# Autodesk Inventor assembly: Team_2374
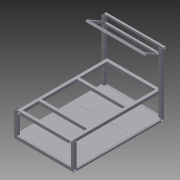
[picture p0: Inventor's stored thumbnail of the model, 180x180]
Saved by Autodesk Inventor 2012 (Build 160160000, 160)
## iProperties
Created: 2011-10-19
Part Number: Team_2374
Document SubType Name: Assembly
Designer: Ian Walters
Mass: 25411.4 g
Surface Area: 59424.9 cm^2
Volume: 9376.89 cm^3
Density: 2.71 g/cm^3
_SolveAssemblyDoc: Frame Generator Solve Assembly
_Version: 15.0.0
Author: Ian Walters
## Documents named in this file (5)
- C:\Users\Ian Walters\Dropbox\CAD Inventor\Preseason Projects\Cart Competition Cart\Team 2374\Team_2374.iam
- C:\Users\Ian Walters\Dropbox\CAD Inventor\Preseason Projects\Cart Competition Cart\Team 2374\Cart Skeleton.ipt
- C:\Users\Ian Walters\Dropbox\CAD Inventor\Preseason Projects\Cart Competition Cart\Team 2374\Team_2374\Frame\Cart Frame.iam
- C:\Users\Ian Walters\Dropbox\CAD Inventor\Preseason Projects\Cart Competition Cart\Team 2374\Bottom Sheet.ipt
- C:\Users\Ian Walters\Dropbox\CAD Inventor\Preseason Projects\Cart Competition Cart\Team 2374\IFI 114 - .1875 x 0.25.ipt
## Components (111 placed, 4 different names)
1. Cart Skeleton:1
2. Cart Frame:1 [sub-assembly] — Mate:1, Mate:2, Mate:3
3. Bottom Sheet:1 — Mate:1, Mate:2, Mate:3, Insert:1, Insert:2, Insert:3, Insert:4
4. IFI 114 - .1875 x 0.25:1 — Insert:1
5. IFI 114 - .1875 x 0.25:2 — Insert:2
6. IFI 114 - .1875 x 0.25:3 — Insert:3
7. IFI 114 - .1875 x 0.25:4 — Insert:4
8. IFI 114 - .1875 x 0.25:5
9. IFI 114 - .1875 x 0.25:6
10. IFI 114 - .1875 x 0.25:7
11. IFI 114 - .1875 x 0.25:8
12. IFI 114 - .1875 x 0.25:9
13. IFI 114 - .1875 x 0.25:10
14. IFI 114 - .1875 x 0.25:11
15. IFI 114 - .1875 x 0.25:12
16. IFI 114 - .1875 x 0.25:13
17. IFI 114 - .1875 x 0.25:14
18. IFI 114 - .1875 x 0.25:15
19. IFI 114 - .1875 x 0.25:16
20. IFI 114 - .1875 x 0.25:17
21. IFI 114 - .1875 x 0.25:18
22. IFI 114 - .1875 x 0.25:19
23. IFI 114 - .1875 x 0.25:20
24. IFI 114 - .1875 x 0.25:21
25. IFI 114 - .1875 x 0.25:22
26. IFI 114 - .1875 x 0.25:23
27. IFI 114 - .1875 x 0.25:24
28. IFI 114 - .1875 x 0.25:25
29. IFI 114 - .1875 x 0.25:26
30. IFI 114 - .1875 x 0.25:27
31. IFI 114 - .1875 x 0.25:28
32. IFI 114 - .1875 x 0.25:29
33. IFI 114 - .1875 x 0.25:30
34. IFI 114 - .1875 x 0.25:31
35. IFI 114 - .1875 x 0.25:32
36. IFI 114 - .1875 x 0.25:33
37. IFI 114 - .1875 x 0.25:34
38. IFI 114 - .1875 x 0.25:35
39. IFI 114 - .1875 x 0.25:36
40. IFI 114 - .1875 x 0.25:37
41. IFI 114 - .1875 x 0.25:38
42. IFI 114 - .1875 x 0.25:39
43. IFI 114 - .1875 x 0.25:40
44. IFI 114 - .1875 x 0.25:41
45. IFI 114 - .1875 x 0.25:42
46. IFI 114 - .1875 x 0.25:43
47. IFI 114 - .1875 x 0.25:44
48. IFI 114 - .1875 x 0.25:45
49. IFI 114 - .1875 x 0.25:46
50. IFI 114 - .1875 x 0.25:47
51. IFI 114 - .1875 x 0.25:48
52. IFI 114 - .1875 x 0.25:49
53. IFI 114 - .1875 x 0.25:50
54. IFI 114 - .1875 x 0.25:51
55. IFI 114 - .1875 x 0.25:52
56. IFI 114 - .1875 x 0.25:53
57. IFI 114 - .1875 x 0.25:54
58. IFI 114 - .1875 x 0.25:55
59. IFI 114 - .1875 x 0.25:56
60. IFI 114 - .1875 x 0.25:57
61. IFI 114 - .1875 x 0.25:58
62. IFI 114 - .1875 x 0.25:59
63. IFI 114 - .1875 x 0.25:60
64. IFI 114 - .1875 x 0.25:61
65. IFI 114 - .1875 x 0.25:62
66. IFI 114 - .1875 x 0.25:63
67. IFI 114 - .1875 x 0.25:64
68. IFI 114 - .1875 x 0.25:65
69. IFI 114 - .1875 x 0.25:66
70. IFI 114 - .1875 x 0.25:67
71. IFI 114 - .1875 x 0.25:68
72. IFI 114 - .1875 x 0.25:69
73. IFI 114 - .1875 x 0.25:70
74. IFI 114 - .1875 x 0.25:71
75. IFI 114 - .1875 x 0.25:72
76. IFI 114 - .1875 x 0.25:73
77. IFI 114 - .1875 x 0.25:74
78. IFI 114 - .1875 x 0.25:75
79. IFI 114 - .1875 x 0.25:76
80. IFI 114 - .1875 x 0.25:77
81. IFI 114 - .1875 x 0.25:78
82. IFI 114 - .1875 x 0.25:79
83. IFI 114 - .1875 x 0.25:80
84. IFI 114 - .1875 x 0.25:81
85. IFI 114 - .1875 x 0.25:82
86. IFI 114 - .1875 x 0.25:83
87. IFI 114 - .1875 x 0.25:84
88. IFI 114 - .1875 x 0.25:85
89. IFI 114 - .1875 x 0.25:86
90. IFI 114 - .1875 x 0.25:87
91. IFI 114 - .1875 x 0.25:88
92. IFI 114 - .1875 x 0.25:89
93. IFI 114 - .1875 x 0.25:90
94. IFI 114 - .1875 x 0.25:91
95. IFI 114 - .1875 x 0.25:92
96. IFI 114 - .1875 x 0.25:93
97. IFI 114 - .1875 x 0.25:94
98. IFI 114 - .1875 x 0.25:95
99. IFI 114 - .1875 x 0.25:96
100. IFI 114 - .1875 x 0.25:97
101. IFI 114 - .1875 x 0.25:98
102. IFI 114 - .1875 x 0.25:99
103. IFI 114 - .1875 x 0.25:100
104. IFI 114 - .1875 x 0.25:101
105. IFI 114 - .1875 x 0.25:102
106. IFI 114 - .1875 x 0.25:103
107. IFI 114 - .1875 x 0.25:104
108. IFI 114 - .1875 x 0.25:105
109. IFI 114 - .1875 x 0.25:106
110. IFI 114 - .1875 x 0.25:107
111. IFI 114 - .1875 x 0.25:108
## Component patterns: (27 elements, first: IFI 114 - .1875 x 0.25:1 + IFI 114 - .1875 x 0.25:2 + IFI 114 - .1875 x 0.25:3 + IFI 114 - .1875 x 0.25:4)
## Relationships (7: Insert 4, Mate 3)
- Mate:1: Cart Frame:1 ↔ Bottom Sheet:1
- Mate:2: Cart Frame:1 ↔ Bottom Sheet:1
- Mate:3: Cart Frame:1 ↔ Bottom Sheet:1
- Insert:1: Bottom Sheet:1 ↔ IFI 114 - .1875 x 0.25:1
- Insert:2: Bottom Sheet:1 ↔ IFI 114 - .1875 x 0.25:2
- Insert:3: Bottom Sheet:1 ↔ IFI 114 - .1875 x 0.25:3
- Insert:4: Bottom Sheet:1 ↔ IFI 114 - .1875 x 0.25:4
